# Autodesk Inventor assembly: Slider_crank_mechanism
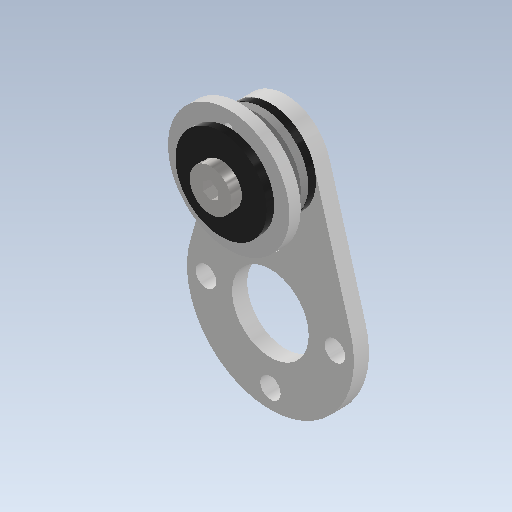
[picture p0: Inventor's stored thumbnail of the model, 512x512]
Saved by Autodesk Inventor 2020.4 (Build 244396000, 396)
## iProperties
Created: 2021-09-06
Part Number: Slider_crank_mechanism
Document SubType Name: Assembly
Designer: Masato Kubotera
Mass: 2.53036 g
Surface Area: 18.5815 cm^2
Volume: 1.13409 cm^3
Density: 2.23118 g/cm^3
Author: Masato Kubotera
## Documents named in this file (8)
- C:\Users\Masato\Documents\Inventor\CIT Brains_Inventor\OpenPlatform_ver3_0\LowerBody\Slider_crank\Slider_crank_mechanism.iam
- C:\Users\Masato\Documents\Inventor\CIT Brains_Inventor\OpenPlatform_ver3_0\LowerBody\Slider_crank\Slider_crank_horn.ipt
- C:\Users\Masato\Documents\Inventor\CIT Brains_Inventor\OpenPlatform_ver3_0\Ready_Made\80F-0603.ipt
- C:\Users\Masato\Documents\Inventor\CIT Brains_Inventor\OpenPlatform_ver3_0\Ready_Made\UUW-0312-10BH.ipt
- C:\Users\Masato\Documents\Inventor\CIT Brains_Inventor\OpenPlatform_ver3_0\Ready_Made\CU-304.5H.ipt
- C:\Users\Masato\Documents\Inventor\CIT Brains_Inventor\OpenPlatform_ver3_0\Ready_Made\S3-07-3W.ipt
- C:\Users\Masato\Documents\Inventor\CIT Brains_Inventor\OpenPlatform_ver3_0\Ready_Made\LFW-0815.ipt
- C:\Users\Masato\Documents\Inventor\CIT Brains_Inventor\OpenPlatform_ver3_0\Ready_Made\Screw\M3-10.ipt
## Components (8 placed, 7 different names)
1. Slider_crank_horn:1 — 挿入:1, 挿入:3
2. 80F-0603:1 — 挿入:2
3. UUW-0312-10BH:1 — 挿入:1, 挿入:2, 挿入:4
4. CU-304.5H:1 — 挿入:4, 挿入:5
5. S3-07-3W:1 — 挿入:3
6. LFW-0815:1 — 挿入:5, 挿入:6
7. UUW-0312-10BH:2 — 挿入:6, 挿入:7
8. M3-10:1 — 挿入:7
## Relationships (7: Insert 7)
- 挿入:1 [Insert]: Slider_crank_horn:1 ↔ UUW-0312-10BH:1
- 挿入:2 [Insert]: 80F-0603:1 ↔ UUW-0312-10BH:1
- 挿入:3 [Insert]: Slider_crank_horn:1 ↔ S3-07-3W:1
- 挿入:4 [Insert]: UUW-0312-10BH:1 ↔ CU-304.5H:1
- 挿入:5 [Insert]: CU-304.5H:1 ↔ LFW-0815:1
- 挿入:6 [Insert]: LFW-0815:1 ↔ UUW-0312-10BH:2
- 挿入:7 [Insert]: UUW-0312-10BH:2 ↔ M3-10:1
